# Autodesk Inventor assembly: 55K stage comparison
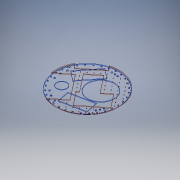
[picture p0: Inventor's stored thumbnail of the model, 180x180]
Saved by Autodesk Inventor 2018 (Build 220112000, 112)
## iProperties
Created: 2018-11-02
Part Number: 55K stage comparison
Document SubType Name: Assembly
Designer: freyja
Author: freyja
## Documents named in this file (4)
- C:\Users\freyja\Documents\Cryorefrigerator\CAD\55K stage comparison.iam
- C:\Users\freyja\Documents\Cryorefrigerator\CAD\existing copper plate 1.ipt
- C:\Users\freyja\Documents\Cryorefrigerator\CAD\mini 55K stage.ipt
- C:\Users\freyja\Documents\Cryorefrigerator\CAD\existing copper plate 2.ipt
## Components (3 placed, 3 different names)
1. mini 55K stage:1 — Mate:1, Mate:2, Mate:3, Mate:4
2. existing copper plate 1:1 — Mate:1, Mate:4
3. existing copper plate 2:1 — Mate:2, Mate:3
## Relationships (4: Mate 4)
- Mate:1: mini 55K stage:1 ↔ existing copper plate 1:1
- Mate:2: mini 55K stage:1 ↔ existing copper plate 2:1
- Mate:3: mini 55K stage:1 ↔ existing copper plate 2:1
- Mate:4: mini 55K stage:1 ↔ existing copper plate 1:1
